# Autodesk Inventor assembly: Pyramid
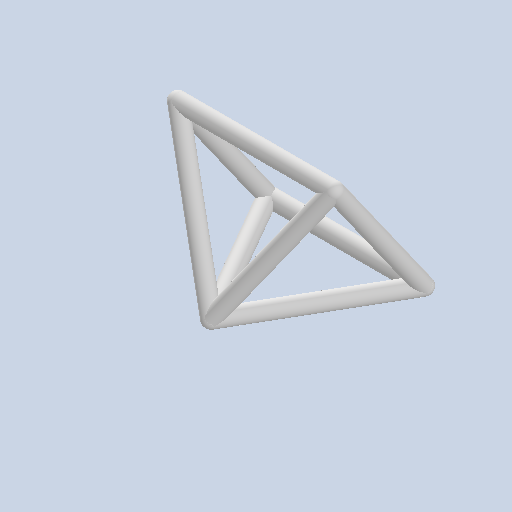
[picture p0: Inventor's stored thumbnail of the model, 512x512]
Saved by Autodesk Inventor 2023 (Build 270158000, 158)
## iProperties
Created: 2023-02-28
Part Number: Pyramid
Document SubType Name: Assembly
Designer: 100KStarsun
Author: 100KStarsun
## Documents named in this file (3)
- C:\Users\100ks\Documents\cwru\Think[Box]\Wire Octohedron\Pyramid.iam
- C:\Users\100ks\Documents\cwru\Think[Box]\Wire Octohedron\Triangle.ipt
- C:\Users\100ks\Documents\cwru\Think[Box]\Wire Octohedron\Square.ipt
## Components (5 placed, 2 different names)
1. Square:1 — Cylindrical:1, Cylindrical:3, Cylindrical:4, Cylindrical:5
2. Triangle:2 — Cylindrical:1, Mate:3
3. Triangle:3 — Cylindrical:3, Mate:1, Mate:2
4. Triangle:4 — Cylindrical:4, Mate:2, Mate:3
5. Triangle:5 — Cylindrical:5, Mate:1
## Relationships (7: CylindricalJoint 4, Mate 3)
- Cylindrical:1: Square:1 ↔ Triangle:2
- Cylindrical:3: Square:1 ↔ Triangle:3
- Cylindrical:4: Square:1 ↔ Triangle:4
- Cylindrical:5: Square:1 ↔ Triangle:5
- Mate:1: Triangle:3 ↔ Triangle:5
- Mate:2: Triangle:3 ↔ Triangle:4
- Mate:3: Triangle:2 ↔ Triangle:4
